# Autodesk Inventor assembly: ServoWithShaftAssembly
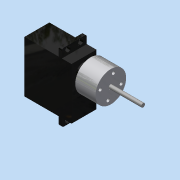
[picture p0: Inventor's stored thumbnail of the model, 180x180]
Saved by Autodesk Inventor 2017 (Build 210142000, 142)
## iProperties
Created: 2016-11-03
Part Number: ServoWithShaftAssembly
Document SubType Name: Assembly
Designer: techn
Author: techn
## Documents named in this file (5)
- D:\OneDrive\Documents\Other Projects\Submarine\CAD\common\3mmShaftToServo\ServoWithShaftAssembly.iam
- D:\OneDrive\Documents\Other Projects\Submarine\CAD\common\HitecServo\HitecServoAssembly.iam
- D:\OneDrive\Documents\Other Projects\Submarine\CAD\common\HitecServo\ServoHornDisc.ipt
- D:\OneDrive\Documents\Other Projects\Submarine\CAD\common\3mmShaftToServo\3mmServoDrivenShaft.ipt
- D:\OneDrive\Documents\Other Projects\Submarine\CAD\common\3mmShaftToServo\1PieceAttachment.ipt
## Components (4 placed, 4 different names)
1. HitecServoAssembly:1 [sub-assembly] — Mate:8, Mate:9
2. ServoHornDisc:1 — Mate:8, Mate:9, Mate:12, Mate:13, Mate:14
3. 3mmServoDrivenShaft:1 — Mate:10, Mate:11
4. 1PieceAttachment:1 — Mate:10, Mate:11, Mate:12, Mate:13, Mate:14
## Relationships (7: Mate 7)
- Mate:8: HitecServoAssembly:1 ↔ ServoHornDisc:1
- Mate:9: HitecServoAssembly:1 ↔ ServoHornDisc:1
- Mate:10: 3mmServoDrivenShaft:1 ↔ 1PieceAttachment:1
- Mate:11: 3mmServoDrivenShaft:1 ↔ 1PieceAttachment:1
- Mate:12: ServoHornDisc:1 ↔ 1PieceAttachment:1
- Mate:13: ServoHornDisc:1 ↔ 1PieceAttachment:1
- Mate:14: ServoHornDisc:1 ↔ 1PieceAttachment:1
